# Autodesk Inventor assembly: PCB Stack Concept V03 02
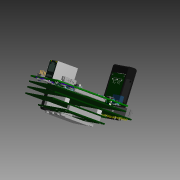
[picture p0: Inventor's stored thumbnail of the model, 180x180]
Saved by Autodesk Inventor 2013 (Build 170138000, 138)
## iProperties
Created: 2014-04-13
Part Number: PCB Stack Concept V03 02
Document SubType Name: Assembly
Designer: spichelh
Author: spichelh
## Documents named in this file (39)
- C:\Users\spichelh\Documents\GitHub\beta-hardware\Enclosure\Version 002\PCB Stack Concept V03 02.iam
- C:\Users\spichelh\Documents\GitHub\beta-hardware\Enclosure\Version 002\Enclosure-Backplate01.ipt
- C:\Users\spichelh\Documents\GitHub\beta-hardware\Enclosure\Version 002\KAC12040.ipt
- C:\Users\spichelh\Documents\GitHub\beta-hardware\Enclosure\Version 002\IRGlass.ipt
- C:\Users\spichelh\Documents\GitHub\beta-hardware\Enclosure\Version 002\Cooler.ipt
- C:\Users\spichelh\Documents\GitHub\beta-hardware\Enclosure\Version 002\Nikon Mount 02.ipt
- C:\Users\spichelh\Documents\GitHub\beta-hardware\Enclosure\Version 002\IOModulePlate01.ipt
- C:\Users\spichelh\Documents\GitHub\beta-hardware\Enclosure\Version 002\PCBModuleLeft01.ipt
- C:\Users\spichelh\Documents\GitHub\beta-hardware\Enclosure\Version 002\IOModulePlate02.ipt
- C:\Users\spichelh\Documents\GitHub\beta-hardware\Enclosure\Version 002\IOModulePlate03.ipt
- C:\Users\spichelh\Documents\GitHub\beta-hardware\Enclosure\Version 002\PCBModuleRight01.ipt
- C:\Users\spichelh\Documents\GitHub\beta-hardware\Enclosure\Version 002\LensBase02.ipt
- C:\Users\spichelh\Documents\GitHub\beta-hardware\Enclosure\Version 002\HexSaver01.ipt
- C:\Users\spichelh\Documents\GitHub\beta-hardware\Enclosure\Version 002\Enclosure03.ipt
- C:\Users\spichelh\Documents\Inventor\Content Center Files\R2013\en-US\ANSI B18.3.1M(1)\ANSI B18.3.1M - M2,5x0,45 x 16(2).ipt
- C:\Users\spichelh\Documents\Inventor\Content Center Files\R2013\en-US\ANSI B18.3.1M(1)\ANSI B18.3.1M - M2,5x0,45 x 35(2).ipt
- C:\Users\spichelh\Documents\GitHub\beta-hardware\Enclosure\Version 002\LensBaseTop01.ipt
- C:\Users\spichelh\Documents\Inventor\Content Center Files\R2013\en-US\ANSI B18.6.3(00)\ANSI B18.6.3 - 3-48 UNC - 0,25(32).ipt
- C:\Users\spichelh\Documents\GitHub\beta-hardware\Enclosure\Version 002\Unmate01.ipt
- C:\Users\spichelh\Documents\GitHub\beta-hardware\Enclosure\Version 002\Parallella.ipt
- C:\Users\spichelh\Documents\GitHub\beta-hardware\Enclosure\Version 002\SFE-Host01.ipt
- C:\Users\spichelh\Documents\GitHub\beta-hardware\Enclosure\Version 002\SFE-ProcessingBoard01.ipt
- C:\Users\spichelh\Documents\GitHub\beta-hardware\Enclosure\Version 002\CMV12000.ipt
- C:\Users\spichelh\Documents\GitHub\beta-hardware\Enclosure\Version 002\Enclosure-Backplate-Variant02.ipt
- C:\Users\spichelh\Documents\GitHub\beta-hardware\Enclosure\Version 002\PCBModuleLeft02.ipt
- C:\Users\spichelh\Documents\GitHub\beta-hardware\Enclosure\Version 002\BetaBoard01.ipt
- C:\Users\spichelh\Documents\GitHub\beta-hardware\Enclosure\Version 002\Imported Components\Zynq_Z010_uZed_F_Prod\Zynq_Z010_uZed_F_Prod.ipt
- C:\Users\spichelh\Documents\GitHub\beta-hardware\Enclosure\Version 002\HighSpeedIOShield01.ipt
- C:\Users\spichelh\Documents\GitHub\beta-hardware\Enclosure\Version 002\AddonPCB01.ipt
- C:\Users\spichelh\Documents\GitHub\beta-hardware\Enclosure\Version 002\F-mount to CMV12k-V04.ipt
- C:\Users\spichelh\Desktop\Imported Components\User Library-Mini Displayport Molex-sd-105081-001\User Library-Mini Displayport Molex-sd-105081-001.ipt
- C:\Users\spichelh\Documents\GitHub\beta-hardware\Enclosure\Version 002\IO-Shield-Sideplate01.ipt
- C:\Users\spichelh\Documents\Inventor\Content Center Files\R2013\en-US\ANSI B18.6.3(25)\ANSI B18.6.3 - 2-56 UNC - 0,125(5).ipt
- C:\Users\spichelh\Documents\GitHub\beta-hardware\Enclosure\Version 002\IO-Shield-Topplate01.ipt
- C:\Users\spichelh\Documents\GitHub\beta-hardware\Enclosure\Version 002\Beta_V2_Top01.ipt
- C:\Users\spichelh\Documents\GitHub\beta-hardware\Enclosure\Version 002\Beta_V2_BendFront01.ipt
- C:\Users\spichelh\Documents\GitHub\beta-hardware\Enclosure\Version 002\PowerPCB01.ipt
- C:\Users\spichelh\Documents\GitHub\beta-hardware\Enclosure\Version 002\Imported Components\Samtec-PCIE-036-02-D-F-TH\Samtec-PCIE-036-02-D-F-TH.ipt
- C:\Users\spichelh\Documents\GitHub\beta-hardware\Enclosure\Version 002\Imported Components\User Library-Mini Displayport Molex-sd-105081-001\User Library-Mini Displayport Molex-sd-105081-001.ipt
## Components (56 placed, 37 different names)
1. Enclosure03:1 — Flush:26, Mate:33, Mate:34, Mate:38, Flush:40, Insert:9, Insert:10, Insert:11, Insert:13, Insert:14, Insert:27, Insert:28, Insert:29, Mate:70, Mate:71, Flush:46, Flush:47
2. Enclosure-Backplate01:1 — Mate:38, Flush:40, Mate:75
3. KAC12040:1 — Mate:72
4. IRGlass:1 — Mate:50, Mate:51, Mate:52
5. Cooler:1 — Mate:145, Flush:120, Flush:121
6. Nikon Mount 02:1 — Mate:31, Mate:32, Insert:3, Mate:50, Mate:51, Mate:52, Insert:18, Insert:19, Insert:20, Insert:21
7. LensBase02:1 — Mate:31, Mate:32, Flush:26, Mate:33, Mate:34, Insert:3, Flush:45
8. IOModulePlate01:1 — Insert:13, Insert:14
9. PCBModuleLeft01:1
10. PCBModuleRight01:1
11. IOModulePlate02:1 — Insert:11
12. IOModulePlate03:1 — Insert:9, Insert:10
13. HexSaver01:1
14. HexSaver01:2
15. HexSaver01:3
16. HexSaver01:4
17. Broached Socket Head Cap Screw - Metric M2,5x0,45 x 16:1 — Insert:18
18. Broached Socket Head Cap Screw - Metric M2,5x0,45 x 16:2 — Insert:19
19. Broached Socket Head Cap Screw - Metric M2,5x0,45 x 16:3 — Insert:20
20. Broached Socket Head Cap Screw - Metric M2,5x0,45 x 16:4 — Insert:21
21. LensBaseTop01:1 — Flush:45, Mate:53, Mate:54
22. Cross Recessed 100° Flat Countersunk Head Machine Screw - Type I - Inch 3-48 UNC x 0,25:2 — Mate:53
23. Cross Recessed 100° Flat Countersunk Head Machine Screw - Type I - Inch 3-48 UNC x 0,25:1 — Mate:54
24. Broached Socket Head Cap Screw - Metric M2,5x0,45 x 35:5 — Mate:55, Mate:70, Mate:71
25. Broached Socket Head Cap Screw - Metric M2,5x0,45 x 35:6 — Insert:27, Mate:59
26. Broached Socket Head Cap Screw - Metric M2,5x0,45 x 35:7 — Insert:28, Mate:66
27. Broached Socket Head Cap Screw - Metric M2,5x0,45 x 35:8 — Insert:29, Mate:57
28. Unmate01:1 — Mate:55
29. Unmate01:2 — Mate:57
30. Unmate01:3 — Mate:59
31. Unmate01:4 — Mate:66
32. Parallella:1
33. SFE-Host01:1 — Mate:72, Mate:73, Flush:48, Flush:49, Mate:76, Flush:50, Flush:51, Mate:130, Flush:121
34. SFE-ProcessingBoard01:1 — Mate:73, Flush:48, Flush:49, Flush:109, Mate:134, Flush:112, Mate:136
35. CMV12000:1 — Mate:76, Flush:50, Flush:51, Mate:91, Mate:92, Mate:93, Mate:129
36. Enclosure-Backplate-Variant02:1 — Mate:75, Flush:46, Flush:47
37. PCBModuleLeft02:1 — Flush:109, Mate:134, Flush:113, Flush:114
38. BetaBoard01:1 — Mate:135, Flush:110, Flush:111, Flush:112, Mate:136, Flush:113, Flush:114, Mate:137, Mate:138, Flush:115, Flush:116, Mate:142, Mate:143, Flush:117, Flush:120
39. Zynq_Z010_uZed_F_Prod:1 — Flush:91, Mate:83, Flush:92, Mate:131, Flush:107, Flush:108
40. HighSpeedIOShield01:1 — Mate:139, Mate:140, Mate:141, Mate:144, Flush:118, Flush:119, Mate:146, Mate:147, Mate:148, Mate:149, Mate:150, Mate:151, Mate:154, Mate:155, Mate:157, Mate:158
41. AddonPCB01:1 — Flush:91, Mate:83, Flush:92
42. F-mount to CMV12k-V04:1 — Mate:91, Mate:92, Mate:93
43. User Library-Mini Displayport Molex-sd-105081-001:1 — Mate:155, Mate:156, Flush:122
44. IO-Shield-Sideplate01:1 — Mate:154, Mate:157, Mate:158
45. Cross Recessed Pan Head Machine Screw - Type IA - Inch No. 2 - 56 - 1/8:1
46. Cross Recessed Pan Head Machine Screw - Type IA - Inch No. 2 - 56 - 1/8:2
47. Cross Recessed Pan Head Machine Screw - Type IA - Inch No. 2 - 56 - 1/8:3
48. Cross Recessed Pan Head Machine Screw - Type IA - Inch No. 2 - 56 - 1/8:4
49. IO-Shield-Topplate01:1 — Mate:146, Mate:147, Mate:151
50. IO-Shield-Topplate01:2 — Mate:148, Mate:149, Mate:150
51. Beta_V2_Top01:1 — Flush:102, Mate:127, Flush:103, Mate:130
52. Beta_V2_BendFront01:1 — Flush:102, Mate:127, Flush:103, Mate:129
53. PowerPCB01:1 — Mate:131, Flush:107, Flush:108, Mate:135, Flush:110, Flush:111, Mate:145
54. Samtec-PCIE-036-02-D-F-TH:1 — Mate:137, Mate:138, Flush:115, Flush:116, Mate:139, Mate:140, Mate:141
55. Samtec-PCIE-036-02-D-F-TH:2 — Mate:142, Mate:143, Flush:117
56. User Library-Mini Displayport Molex-sd-105081-001:3 — Mate:144, Flush:118, Flush:119, Mate:156, Flush:122
## Relationships (93: Mate 51, Flush 29, Insert 13)
- Mate:31: Nikon Mount 02:1 ↔ LensBase02:1
- Mate:32: Nikon Mount 02:1 ↔ LensBase02:1
- Flush:26: Enclosure03:1 ↔ LensBase02:1
- Mate:33: Enclosure03:1 ↔ LensBase02:1
- Mate:34: Enclosure03:1 ↔ LensBase02:1
- Insert:3: Nikon Mount 02:1 ↔ LensBase02:1
- Mate:38 (3 mm): Enclosure03:1 ↔ Enclosure-Backplate01:1
- Flush:40: Enclosure03:1 ↔ Enclosure-Backplate01:1
- Insert:9: Enclosure03:1 ↔ IOModulePlate03:1
- Insert:10: Enclosure03:1 ↔ IOModulePlate03:1
- Insert:11: Enclosure03:1 ↔ IOModulePlate02:1
- Insert:13: Enclosure03:1 ↔ IOModulePlate01:1
- Insert:14: Enclosure03:1 ↔ IOModulePlate01:1
- Mate:50: IRGlass:1 ↔ Nikon Mount 02:1
- Mate:51 (0.5 mm): IRGlass:1 ↔ Nikon Mount 02:1
- Mate:52 (0.5 mm): IRGlass:1 ↔ Nikon Mount 02:1
- Flush:45: LensBase02:1 ↔ LensBaseTop01:1
- Mate:55: Broached Socket Head Cap Screw - Metric M2,5x0,45 x 35:5 ↔ Unmate01:1
- Mate:57: Broached Socket Head Cap Screw - Metric M2,5x0,45 x 35:8 ↔ Unmate01:2
- Mate:59: Broached Socket Head Cap Screw - Metric M2,5x0,45 x 35:6 ↔ Unmate01:3
- Mate:66: Broached Socket Head Cap Screw - Metric M2,5x0,45 x 35:7 ↔ Unmate01:4
- Mate:70: Enclosure03:1 ↔ Broached Socket Head Cap Screw - Metric M2,5x0,45 x 35:5
- Mate:71: Enclosure03:1 ↔ Broached Socket Head Cap Screw - Metric M2,5x0,45 x 35:5
- Mate:72: KAC12040:1 ↔ SFE-Host01:1
- Mate:73: SFE-Host01:1 ↔ SFE-ProcessingBoard01:1
- Mate:75 (10 mm): Enclosure-Backplate01:1 ↔ Enclosure-Backplate-Variant02:1
- Flush:46: Enclosure03:1 ↔ Enclosure-Backplate-Variant02:1
- Flush:47: Enclosure03:1 ↔ Enclosure-Backplate-Variant02:1
- Flush:48: SFE-Host01:1 ↔ SFE-ProcessingBoard01:1
- Flush:49: SFE-Host01:1 ↔ SFE-ProcessingBoard01:1
- Mate:76 (3 mm): SFE-Host01:1 ↔ CMV12000:1
- Flush:50 (6 mm): SFE-Host01:1 ↔ CMV12000:1
- Flush:51 (11.75 mm): SFE-Host01:1 ↔ CMV12000:1
- Flush:91: Zynq_Z010_uZed_F_Prod:1 ↔ AddonPCB01:1
- Mate:83: Zynq_Z010_uZed_F_Prod:1 ↔ AddonPCB01:1
- Flush:92: Zynq_Z010_uZed_F_Prod:1 ↔ AddonPCB01:1
- Mate:91: CMV12000:1 ↔ F-mount to CMV12k-V04:1
- Mate:92: CMV12000:1 ↔ F-mount to CMV12k-V04:1
- Mate:93: CMV12000:1 ↔ F-mount to CMV12k-V04:1
- Flush:102: Beta_V2_Top01:1 ↔ Beta_V2_BendFront01:1
- Mate:127: Beta_V2_Top01:1 ↔ Beta_V2_BendFront01:1
- Flush:103: Beta_V2_Top01:1 ↔ Beta_V2_BendFront01:1
- Mate:129 (3 mm): CMV12000:1 ↔ Beta_V2_BendFront01:1
- Mate:130 (2 mm): SFE-Host01:1 ↔ Beta_V2_Top01:1
- Mate:131 (5 mm): Zynq_Z010_uZed_F_Prod:1 ↔ PowerPCB01:1
- Flush:107: Zynq_Z010_uZed_F_Prod:1 ↔ PowerPCB01:1
- Flush:108: Zynq_Z010_uZed_F_Prod:1 ↔ PowerPCB01:1
- Flush:109: SFE-ProcessingBoard01:1 ↔ PCBModuleLeft02:1
- Mate:134 (1 mm): SFE-ProcessingBoard01:1 ↔ PCBModuleLeft02:1
- Mate:135 (5 mm): BetaBoard01:1 ↔ PowerPCB01:1
- Flush:110: BetaBoard01:1 ↔ PowerPCB01:1
- Flush:111: BetaBoard01:1 ↔ PowerPCB01:1
- Flush:112: SFE-ProcessingBoard01:1 ↔ BetaBoard01:1
- Mate:136: SFE-ProcessingBoard01:1 ↔ BetaBoard01:1
- Flush:113: PCBModuleLeft02:1 ↔ BetaBoard01:1
- Flush:114: PCBModuleLeft02:1 ↔ BetaBoard01:1
- Mate:137: BetaBoard01:1 ↔ Samtec-PCIE-036-02-D-F-TH:1
- Mate:138: BetaBoard01:1 ↔ Samtec-PCIE-036-02-D-F-TH:1
- Flush:115: BetaBoard01:1 ↔ Samtec-PCIE-036-02-D-F-TH:1
- Flush:116 (1.4908 mm): BetaBoard01:1 ↔ Samtec-PCIE-036-02-D-F-TH:1
- Mate:139: HighSpeedIOShield01:1 ↔ Samtec-PCIE-036-02-D-F-TH:1
- Mate:140: HighSpeedIOShield01:1 ↔ Samtec-PCIE-036-02-D-F-TH:1
- Mate:141: HighSpeedIOShield01:1 ↔ Samtec-PCIE-036-02-D-F-TH:1
- Mate:142: BetaBoard01:1 ↔ Samtec-PCIE-036-02-D-F-TH:2
- Mate:143: BetaBoard01:1 ↔ Samtec-PCIE-036-02-D-F-TH:2
- Flush:117 (2.0906 mm): BetaBoard01:1 ↔ Samtec-PCIE-036-02-D-F-TH:2
- Mate:144: HighSpeedIOShield01:1 ↔ User Library-Mini Displayport Molex-sd-105081-001:3
- Flush:118 (5 mm): HighSpeedIOShield01:1 ↔ User Library-Mini Displayport Molex-sd-105081-001:3
- Flush:119 (5 mm): HighSpeedIOShield01:1 ↔ User Library-Mini Displayport Molex-sd-105081-001:3
- Mate:145: Cooler:1 ↔ PowerPCB01:1
- Flush:120 (30 mm): Cooler:1 ↔ BetaBoard01:1
- Mate:146: HighSpeedIOShield01:1 ↔ IO-Shield-Topplate01:1
- Mate:147: HighSpeedIOShield01:1 ↔ IO-Shield-Topplate01:1
- Mate:148: HighSpeedIOShield01:1 ↔ IO-Shield-Topplate01:2
- Mate:149: HighSpeedIOShield01:1 ↔ IO-Shield-Topplate01:2
- Mate:150: HighSpeedIOShield01:1 ↔ IO-Shield-Topplate01:2
- Mate:151: HighSpeedIOShield01:1 ↔ IO-Shield-Topplate01:1
- Mate:154: HighSpeedIOShield01:1 ↔ IO-Shield-Sideplate01:1
- Mate:155: HighSpeedIOShield01:1 ↔ User Library-Mini Displayport Molex-sd-105081-001:1
- Mate:156 (1 mm): User Library-Mini Displayport Molex-sd-105081-001:1 ↔ User Library-Mini Displayport Molex-sd-105081-001:3
- Flush:121 (2 mm): Cooler:1 ↔ SFE-Host01:1
- Mate:157: HighSpeedIOShield01:1 ↔ IO-Shield-Sideplate01:1
- Mate:158: HighSpeedIOShield01:1 ↔ IO-Shield-Sideplate01:1
- Flush:122: User Library-Mini Displayport Molex-sd-105081-001:1 ↔ User Library-Mini Displayport Molex-sd-105081-001:3
- Insert:18: Nikon Mount 02:1 ↔ Broached Socket Head Cap Screw - Metric M2,5x0,45 x 16:1
- Insert:19: Nikon Mount 02:1 ↔ Broached Socket Head Cap Screw - Metric M2,5x0,45 x 16:2
- Insert:20: Nikon Mount 02:1 ↔ Broached Socket Head Cap Screw - Metric M2,5x0,45 x 16:3
- Insert:21: Nikon Mount 02:1 ↔ Broached Socket Head Cap Screw - Metric M2,5x0,45 x 16:4
- Mate:53: LensBaseTop01:1 ↔ Cross Recessed 100° Flat Countersunk Head Machine Screw - Type I - Inch 3-48 UNC x 0,25:2
- Mate:54: LensBaseTop01:1 ↔ Cross Recessed 100° Flat Countersunk Head Machine Screw - Type I - Inch 3-48 UNC x 0,25:1
- Insert:27: Enclosure03:1 ↔ Broached Socket Head Cap Screw - Metric M2,5x0,45 x 35:6
- Insert:28: Enclosure03:1 ↔ Broached Socket Head Cap Screw - Metric M2,5x0,45 x 35:7
- Insert:29: Enclosure03:1 ↔ Broached Socket Head Cap Screw - Metric M2,5x0,45 x 35:8
